# Autodesk Inventor assembly: S2_Gantry_500
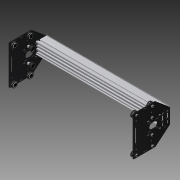
[picture p0: Inventor's stored thumbnail of the model, 180x180]
Saved by Autodesk Inventor 2014 (Build 180170000, 170)
## iProperties
Created: 2013-09-18
Part Number: S2_Gantry_500
Document SubType Name: Assembly
Designer: Edward
Author: Edward
## Documents named in this file (6)
- C:\Users\Edward\Documents\Vault\Designs\Shapeoko_v2\v2_final\assemblies\S2_Gantry_500.iam
- C:\Users\Edward\Documents\Vault\Designs\Shapeoko_v2\v2_final\plate_assembly_stacked.iam
- C:\Users\Edward\Documents\Vault\Designs\Shapeoko_v2\v2_final\belt_clip_assembly.iam
- C:\Users\Edward\Documents\Vault\Designs\Shapeoko_v2\v2_final\25286-02.ipt
- C:\Users\Edward\Documents\Vault\Designs\Shapeoko_v2\v2_final\25287-02.ipt
- C:\Users\Edward\Documents\Vault\Designs\Shapeoko_v2\v2_final\25142-XX500.ipt
## Components (22 placed, 5 different names)
1. 25142-XX500:1 — Flush:6, Flush:7
2. plate_assembly_stacked:1 [sub-assembly] — Flush:6
3. plate_assembly_stacked:2 [sub-assembly] — Mate:9
4. belt_clip_assembly:1 [sub-assembly]
5. belt_clip_assembly:2 [sub-assembly]
6. 25286-02:1
7. 25287-02:1
8. 25286-02:2
9. 25287-02:2
10. 25286-02:3
11. 25287-02:3
12. 25286-02:4
13. 25287-02:4
14. 25142-XX500:2 — Mate:9, Flush:7, Insert:11, Insert:13, Insert:16, Insert:17
15. 25286-02:5
16. 25287-02:5 — Insert:11
17. 25286-02:6
18. 25287-02:6 — Insert:13
19. 25286-02:7
20. 25287-02:7 — Insert:17
21. 25286-02:8
22. 25287-02:8 — Insert:16
## Relationships (31: Insert 17, Mate 8, Flush 6)
- [Flush]: plate_assembly_stacked:1 ↔ plate_assembly_stacked:2
- [Mate] (500 mm): plate_assembly_stacked:1 ↔ plate_assembly_stacked:2
- [Mate]: 25142-XX500:1 ↔ plate_assembly_stacked:1
- [Mate]: 25142-XX500:1 ↔ plate_assembly_stacked:2
- [Flush]: 25142-XX500:1 ↔ plate_assembly_stacked:2
- [Insert]: 25142-XX500:1 ↔ plate_assembly_stacked:2
- [Mate]: 25142-XX500:1 ↔ belt_clip_assembly:1
- [Flush] (3 mm): 25142-XX500:1 ↔ belt_clip_assembly:1
- [Mate]: plate_assembly_stacked:1 ↔ belt_clip_assembly:1
- [Mate]: 25142-XX500:1 ↔ belt_clip_assembly:2
- [Flush] (3 mm): 25142-XX500:1 ↔ belt_clip_assembly:2
- [Mate]: plate_assembly_stacked:2 ↔ belt_clip_assembly:2
- [Insert]: 25286-02:1 ↔ 25287-02:1
- [Insert]: 25286-02:2 ↔ 25287-02:2
- [Insert] (3.4163 mm): 25142-XX500:1 ↔ 25287-02:1
- [Insert] (3.4163 mm): 25142-XX500:1 ↔ 25287-02:2
- [Insert]: 25286-02:3 ↔ 25287-02:3
- [Insert]: 25286-02:4 ↔ 25287-02:4
- [Insert] (3.4163 mm): 25142-XX500:1 ↔ 25287-02:4
- [Insert] (3.4163 mm): 25142-XX500:1 ↔ 25287-02:3
- Flush:6: 25142-XX500:1 ↔ plate_assembly_stacked:1
- Mate:9: plate_assembly_stacked:2 ↔ 25142-XX500:2
- Flush:7: 25142-XX500:1 ↔ 25142-XX500:2
- [Insert]: 25286-02:5 ↔ 25287-02:5
- Insert:11 (2.36 mm): 25142-XX500:2 ↔ 25287-02:5
- [Insert]: 25286-02:6 ↔ 25287-02:6
- Insert:13 (2.36 mm): 25142-XX500:2 ↔ 25287-02:6
- [Insert]: 25286-02:7 ↔ 25287-02:7
- [Insert]: 25286-02:8 ↔ 25287-02:8
- Insert:16 (2.36 mm): 25142-XX500:2 ↔ 25287-02:8
- Insert:17 (2.36 mm): 25142-XX500:2 ↔ 25287-02:7
## Named parameters: d101_d55_d51 = 0 mm, d102_d55_d51 = 0 mm, d105_d55_d51 = 0 mm, d106_d55_d51 = 0 mm, d26_d101_d55_d51 = 0 mm, d28_d101_d55_d51 = 0 mm, d30_d101_d55_d51 = 0 mm, d31_d101_d55_d51 = 0 mm
